# Autodesk Inventor assembly: MBD_RL_l4
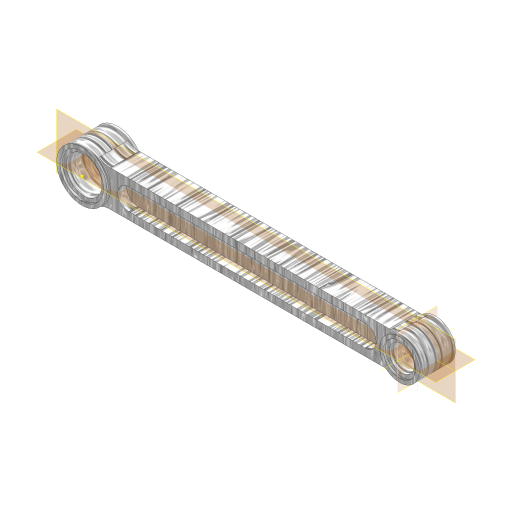
[picture p0: Inventor's stored thumbnail of the model, 512x512]
Saved by Autodesk Inventor 2023 (Build 270158000, 158)
## iProperties
Created: 2022-06-22
Part Number: MBD_RL_l4
Document SubType Name: Assembly
Designer: BioRoLaT470S
Mass: 14.9703 g
Surface Area: 50.0483 cm^2
Volume: 5.32751 cm^3
Density: 2.81 g/cm^3
Author: BioRoLaT470S
## Documents named in this file (2)
- C:\Users\guanlunlu\Desktop\MBD_CORGI\CAD\MBD_RL_l4.iam
- C:\Users\guanlunlu\Desktop\MBD_CORGI\R100_properties\組合檔_v4\I4_v2.ipt
## Components (1 placed, 1 different names)
1. I4_v2:1 — Mate:1, Flush:1, Flush:2
## Relationships (3: Flush 2, Mate 1)
- Mate:1: I4_v2:1
- Flush:1: I4_v2:1
- Flush:2: I4_v2:1
